# Autodesk Inventor assembly: tower1
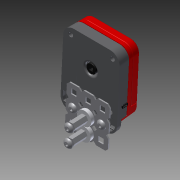
[picture p0: Inventor's stored thumbnail of the model, 180x180]
Saved by Autodesk Inventor 2014 SP1 (Build 180222100, 222)
## iProperties
Created: 2013-08-29
Part Number: tower1
Document SubType Name: Assembly
Designer: Ryan
Author: Ryan
## Documents named in this file (7)
- C:\Users\Ryan\Desktop\pack and go\Workspaces\Workspace\toss up 1st A bot\toss up tower\encoder metal assembly.iam
- C:\Users\Ryan\Desktop\pack and go\Workspaces\Workspace\lib\Aperture VEX CAD Library\Hardware\8-32\8-32_.375.ipt
- C:\Users\Ryan\Desktop\pack and go\Workspaces\Workspace\lib\Aperture VEX CAD Library\Standoffs\BEAM-0500.ipt
- C:\Users\Ryan\Desktop\pack and go\Workspaces\Workspace\lib\Aperture VEX CAD Library\Metal\Plate\3 x 3.ipt
- C:\Users\Ryan\Desktop\pack and go\Workspaces\Workspace\lib\Aperture VEX CAD Library\Spacers\SPACER-0500-0125.ipt
- C:\Users\Ryan\Desktop\pack and go\Workspaces\Workspace\lib\Super Sonic Sparks VEX CAD Library\Motors & Sensors\Optical Shaft (Quadrature) Encoder.iam
- C:\Users\Ryan\Desktop\pack and go\Workspaces\Workspace\lib\Aperture VEX CAD Library\Hardware\8-32\8-32 nylock.ipt
## Components (14 placed, 6 different names)
1. 3 x 3:1 — Mate:72, Mate:73, Mate:75, Mate:76, Mate:77, Flush:6, Mate:82, Mate:83, Mate:84, Mate:88
2. Optical Shaft (Quadrature) Encoder:1 [sub-assembly] — Mate:73, Flush:6, Mate:79, Mate:85, Mate:88
3. 8-32_.375:9 — Mate:74, Mate:75, Mate:76, Mate:77
4. 8-32_.375:10 — Mate:79, Mate:80
5. 8-32_.375:7 — Mate:68, Mate:87
6. BEAM-0500:6 — Mate:68, Mate:70, Mate:71, Mate:87
7. SPACER-0500-0125:1 — Mate:70, Mate:71, Mate:72, Mate:74
8. 8-32_.375:8
9. BEAM-0500:7
10. SPACER-0500-0125:2 — Mate:80
11. 8-32_.375:11 — Mate:82, Mate:83, Mate:84, Mate:86
12. 8-32 nylock:1 — Mate:85, Mate:86
13. 8-32_.375:12
14. 8-32 nylock:2
## Component patterns: (2 elements, first: 8-32_.375:7 + BEAM-0500:6 + SPACER-0500-0125:1), (2 elements, first: 8-32_.375:11 + 8-32 nylock:1)
## Relationships (19: Mate 18, Flush 1)
- Mate:68: 8-32_.375:7 ↔ BEAM-0500:6
- Mate:70: BEAM-0500:6 ↔ SPACER-0500-0125:1
- Mate:71: BEAM-0500:6 ↔ SPACER-0500-0125:1
- Mate:72: 3 x 3:1 ↔ SPACER-0500-0125:1
- Mate:73: 3 x 3:1 ↔ Optical Shaft (Quadrature) Encoder:1
- Mate:74: 8-32_.375:9 ↔ SPACER-0500-0125:1
- Mate:75: 3 x 3:1 ↔ 8-32_.375:9
- Mate:76 (2.3114 mm): 3 x 3:1 ↔ 8-32_.375:9
- Mate:77 (2.3114 mm): 3 x 3:1 ↔ 8-32_.375:9
- Flush:6 (0.0635 mm): 3 x 3:1 ↔ Optical Shaft (Quadrature) Encoder:1
- Mate:79: Optical Shaft (Quadrature) Encoder:1 ↔ 8-32_.375:10
- Mate:80: 8-32_.375:10 ↔ SPACER-0500-0125:2
- Mate:82: 3 x 3:1 ↔ 8-32_.375:11
- Mate:83 (2.3114 mm): 3 x 3:1 ↔ 8-32_.375:11
- Mate:84 (2.3114 mm): 3 x 3:1 ↔ 8-32_.375:11
- Mate:85: Optical Shaft (Quadrature) Encoder:1 ↔ 8-32 nylock:1
- Mate:86: 8-32_.375:11 ↔ 8-32 nylock:1
- Mate:87 (1.5875 mm): 8-32_.375:7 ↔ BEAM-0500:6
- Mate:88 (2.3114 mm): 3 x 3:1 ↔ Optical Shaft (Quadrature) Encoder:1
## Named parameters: q = 2.3114 mm, encoder = 0.0635 mm
